# Autodesk Inventor assembly: Assembly2
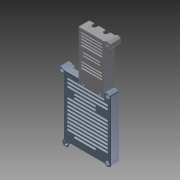
[picture p0: Inventor's stored thumbnail of the model, 180x180]
Saved by Autodesk Inventor 2012 (Build 160160000, 160)
## iProperties
Created: 2018-03-05
Part Number: Assembly2
Document SubType Name: Assembly
Designer: kanu
Author: kanu
## Documents named in this file (3)
- C:\Users\kanu\Documents\Inventor\mi-streamer-box\Assembly2.iam
- C:\Users\kanu\Documents\Inventor\mi-streamer-box\audio case base v2.ipt
- C:\Users\kanu\Documents\Inventor\mi-streamer-box\case add on sdr botom.ipt
## Components (2 placed, 2 different names)
1. audio case base v2:1 — Mate:1, Mate:2, Mate:3
2. case add on sdr botom:1 — Mate:1, Mate:2, Mate:3
## Relationships (3: Mate 3)
- Mate:1: audio case base v2:1 ↔ case add on sdr botom:1
- Mate:2: audio case base v2:1 ↔ case add on sdr botom:1
- Mate:3 (0.1 mm): audio case base v2:1 ↔ case add on sdr botom:1
